# Autodesk Inventor assembly: Assembly1
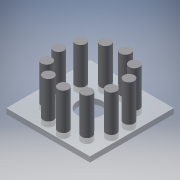
[picture p0: Inventor's stored thumbnail of the model, 180x180]
Saved by Autodesk Inventor 2019 (Build 230136000, 136)
## iProperties
Created: 2019-05-17
Part Number: Assembly1
Document SubType Name: Assembly
Designer: Alex Jones
Author: Alex Jones
## Documents named in this file (3)
- C:\Users\Alex Jones\Documents\Inventor\cylcoid\Assembly1.iam
- C:\Users\Alex Jones\Documents\Inventor\cylcoid\basePlate.ipt
- C:\Users\Alex Jones\Documents\Inventor\cylcoid\rodStandin.ipt
## Components (12 placed, 2 different names)
1. basePlate:1 — Mate:1, Mate:2, Mate:3, Mate:4, Mate:5, Mate:6, Mate:7, Mate:8, Mate:9, Mate:10, Mate:11, Flush:11
2. rodStandin:2 — Mate:11, Flush:9, Flush:10
3. rodStandin:3 — Mate:10, Flush:10
4. rodStandin:4 — Mate:8, Flush:1, Flush:2, Flush:11
5. rodStandin:5 — Mate:9, Flush:1
6. rodStandin:6 — Mate:7, Flush:2, Flush:3
7. rodStandin:7 — Mate:6, Flush:3, Flush:4
8. rodStandin:8 — Mate:5, Flush:4, Flush:5
9. rodStandin:9 — Mate:4, Flush:5, Flush:6
10. rodStandin:10 — Mate:3, Flush:6, Flush:7
11. rodStandin:11 — Mate:2, Flush:7, Flush:8
12. rodStandin:12 — Mate:1, Flush:8, Flush:9
## Relationships (22: Mate 11, Flush 11)
- Mate:1: basePlate:1 ↔ rodStandin:12
- Mate:2: basePlate:1 ↔ rodStandin:11
- Mate:3: basePlate:1 ↔ rodStandin:10
- Mate:4: basePlate:1 ↔ rodStandin:9
- Mate:5: basePlate:1 ↔ rodStandin:8
- Mate:6: basePlate:1 ↔ rodStandin:7
- Mate:7: basePlate:1 ↔ rodStandin:6
- Mate:8: basePlate:1 ↔ rodStandin:4
- Mate:9: basePlate:1 ↔ rodStandin:5
- Mate:10: basePlate:1 ↔ rodStandin:3
- Mate:11: basePlate:1 ↔ rodStandin:2
- Flush:1: rodStandin:4 ↔ rodStandin:5
- Flush:2: rodStandin:4 ↔ rodStandin:6
- Flush:3: rodStandin:6 ↔ rodStandin:7
- Flush:4: rodStandin:7 ↔ rodStandin:8
- Flush:5: rodStandin:8 ↔ rodStandin:9
- Flush:6: rodStandin:9 ↔ rodStandin:10
- Flush:7: rodStandin:10 ↔ rodStandin:11
- Flush:8: rodStandin:11 ↔ rodStandin:12
- Flush:9: rodStandin:2 ↔ rodStandin:12
- Flush:10: rodStandin:2 ↔ rodStandin:3
- Flush:11: basePlate:1 ↔ rodStandin:4
